# Autodesk Inventor assembly: MecanumWheelFullForVexmotor
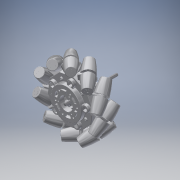
[picture p0: Inventor's stored thumbnail of the model, 180x180]
Saved by Autodesk Inventor 2017 (Build 210142000, 142)
## iProperties
Created: 2017-12-02
Part Number: MecanumWheelFullForVexmotor
Document SubType Name: Assembly
Designer: User
Author: User
## Documents named in this file (5)
- C:\Robotics\CAD\2017-18_CAD\Prototypes\MecanumWheelFullForVexmotor.iam
- C:\Robotics\CAD\COTSParts\Vex\6inchMecanumRight217-2586-STEP\6inchMecanumRight217-2586.20121203.ipt
- C:\Robotics\CAD\COTSParts\Rev\REV-41-1147HexHub.ipt
- C:\Robotics\CAD\COTSParts\Rev\REV-41-1349.ipt
- C:\Robotics\CAD\2017-18_CAD\Prototypes\NewMechanumWheelHub.ipt
## Components (4 placed, 4 different names)
1. 6inchMecanumRight217-2586.20121203:1 — Mate:23, Insert:1, Insert:2
2. REV-41-1147HexHub:2 — Mate:24, Insert:3, Mate:25
3. REV-41-1349:1
4. NewMechanumWheelHub:2 — Mate:23, Insert:1, Insert:2, Mate:24, Insert:3, Mate:25
## Relationships (6: Mate 3, Insert 3)
- Mate:23: 6inchMecanumRight217-2586.20121203:1 ↔ NewMechanumWheelHub:2
- Insert:1: 6inchMecanumRight217-2586.20121203:1 ↔ NewMechanumWheelHub:2
- Insert:2: 6inchMecanumRight217-2586.20121203:1 ↔ NewMechanumWheelHub:2
- Mate:24: REV-41-1147HexHub:2 ↔ NewMechanumWheelHub:2
- Insert:3: REV-41-1147HexHub:2 ↔ NewMechanumWheelHub:2
- Mate:25: REV-41-1147HexHub:2 ↔ NewMechanumWheelHub:2
